# Autodesk Inventor assembly: Pneumatic Wheel Assembly
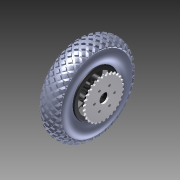
[picture p0: Inventor's stored thumbnail of the model, 180x180]
Saved by Autodesk Inventor 2013 (Build 170138000, 138)
## iProperties
Created: 2013-08-13
Part Number: Pneumatic Wheel Assembly
Document SubType Name: Assembly
Designer: Creo
Author: Creo
## Documents named in this file (5)
- E:\Pneumatic Wheel Assembly.iam
- E:\Imported Components\PneumaticWheel_am-0970\PneumaticWheel_am-0970.iam
- E:\550 Sprocket Spacer (am-0651).ipt
- E:\AM-0146\AM-0146 S35-30 Sprocket.ipt
- C:\Users\Creo\Documents\Inventor\Content Center Files\R2013\en-US\ANSI B18.6.3(24)\ANSI B18.6.3 - 4-40 UNC - 1(4A).ipt
## Components (9 placed, 4 different names)
1. PneumaticWheel_am-0970:1 [sub-assembly] — Mate:1, Mate:2, Mate:3
2. 550 Sprocket Spacer (am-0651):1 — Mate:1, Mate:2, Mate:3, Mate:4, Mate:5, Mate:6, Mate:7
3. AM-0146 S35-30 Sprocket:1 — Mate:4, Mate:5, Mate:6, Mate:7, Mate:8, Mate:9, Mate:10, Mate:11, Mate:12, Mate:13, Mate:14, Mate:15, Mate:16, Mate:17, Mate:18, Mate:19
4. Cross Recessed Pan Head Machine Screw - Type I - Inch No. 4 - 40 - 1:1 — Mate:14, Mate:15
5. Cross Recessed Pan Head Machine Screw - Type I - Inch No. 4 - 40 - 1:2 — Mate:16, Mate:18
6. Cross Recessed Pan Head Machine Screw - Type I - Inch No. 4 - 40 - 1:3 — Mate:17, Mate:19
7. Cross Recessed Pan Head Machine Screw - Type I - Inch No. 4 - 40 - 1:4 — Mate:12, Mate:13
8. Cross Recessed Pan Head Machine Screw - Type I - Inch No. 4 - 40 - 1:5 — Mate:8, Mate:9
9. Cross Recessed Pan Head Machine Screw - Type I - Inch No. 4 - 40 - 1:6 — Mate:10, Mate:11
## Relationships (19: Mate 19)
- Mate:1: PneumaticWheel_am-0970:1 ↔ 550 Sprocket Spacer (am-0651):1
- Mate:2: PneumaticWheel_am-0970:1 ↔ 550 Sprocket Spacer (am-0651):1
- Mate:3: PneumaticWheel_am-0970:1 ↔ 550 Sprocket Spacer (am-0651):1
- Mate:4: 550 Sprocket Spacer (am-0651):1 ↔ AM-0146 S35-30 Sprocket:1
- Mate:5: 550 Sprocket Spacer (am-0651):1 ↔ AM-0146 S35-30 Sprocket:1
- Mate:6: 550 Sprocket Spacer (am-0651):1 ↔ AM-0146 S35-30 Sprocket:1
- Mate:7: 550 Sprocket Spacer (am-0651):1 ↔ AM-0146 S35-30 Sprocket:1
- Mate:8: AM-0146 S35-30 Sprocket:1 ↔ Cross Recessed Pan Head Machine Screw - Type I - Inch No. 4 - 40 - 1:5
- Mate:9: AM-0146 S35-30 Sprocket:1 ↔ Cross Recessed Pan Head Machine Screw - Type I - Inch No. 4 - 40 - 1:5
- Mate:10: AM-0146 S35-30 Sprocket:1 ↔ Cross Recessed Pan Head Machine Screw - Type I - Inch No. 4 - 40 - 1:6
- Mate:11: AM-0146 S35-30 Sprocket:1 ↔ Cross Recessed Pan Head Machine Screw - Type I - Inch No. 4 - 40 - 1:6
- Mate:12: AM-0146 S35-30 Sprocket:1 ↔ Cross Recessed Pan Head Machine Screw - Type I - Inch No. 4 - 40 - 1:4
- Mate:13: AM-0146 S35-30 Sprocket:1 ↔ Cross Recessed Pan Head Machine Screw - Type I - Inch No. 4 - 40 - 1:4
- Mate:14: AM-0146 S35-30 Sprocket:1 ↔ Cross Recessed Pan Head Machine Screw - Type I - Inch No. 4 - 40 - 1:1
- Mate:15: AM-0146 S35-30 Sprocket:1 ↔ Cross Recessed Pan Head Machine Screw - Type I - Inch No. 4 - 40 - 1:1
- Mate:16: AM-0146 S35-30 Sprocket:1 ↔ Cross Recessed Pan Head Machine Screw - Type I - Inch No. 4 - 40 - 1:2
- Mate:17: AM-0146 S35-30 Sprocket:1 ↔ Cross Recessed Pan Head Machine Screw - Type I - Inch No. 4 - 40 - 1:3
- Mate:18: AM-0146 S35-30 Sprocket:1 ↔ Cross Recessed Pan Head Machine Screw - Type I - Inch No. 4 - 40 - 1:2
- Mate:19: AM-0146 S35-30 Sprocket:1 ↔ Cross Recessed Pan Head Machine Screw - Type I - Inch No. 4 - 40 - 1:3
